# Autodesk Inventor assembly: 110033226_iam_14_內城堡
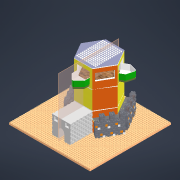
[picture p0: Inventor's stored thumbnail of the model, 180x180]
Saved by Autodesk Inventor 2022 (Build 260153000, 153)
## iProperties
Created: 2022-07-01
Part Number: 110033226_iam_14_內城堡
Document SubType Name: Assembly
Designer: User
Author: User
## Documents named in this file (4)
- D:\D-disk\pomelo\大一\下學期\機械設計製圖\1100332260_LEGOproj_沒有公主城堡\110033226_iam_14_內城堡.iam
- D:\D-disk\pomelo\大一\下學期\機械設計製圖\1100332260_LEGOproj_沒有公主城堡\110033226_ipt_54_內城堡底座.ipt
- D:\D-disk\pomelo\大一\下學期\機械設計製圖\1100332260_LEGOproj_沒有公主城堡\110033226_ipt_54_內城堡中柱.ipt
- D:\D-disk\pomelo\大一\下學期\機械設計製圖\1100332260_LEGOproj_沒有公主城堡\110033226_ipt_34_中心城堡圍牆.ipt
## Components (14 placed, 3 different names)
1. 110033226_ipt_54_內城堡底座:1 — 貼合:1, 貼合:2, 貼合:3, 貼合:4, 角度:1, 貼合:5, 貼合:9, 貼合:12, 貼合:15, 貼合:18
2. 110033226_ipt_54_內城堡中柱:1 — 貼合:4, 角度:1, 貼合:5, 貼合:10, 貼合:11, 貼合:13, 貼合:14, 貼合:16, 貼合:17, 貼合:19, 貼合:20
3. 110033226_ipt_34_中心城堡圍牆:2 — 貼合:9, 貼合:10, 貼合:11
4. 110033226_ipt_34_中心城堡圍牆:5
5. 110033226_ipt_34_中心城堡圍牆:6
6. 110033226_ipt_34_中心城堡圍牆:1 — 貼合:12, 貼合:13, 貼合:14
7. 110033226_ipt_34_中心城堡圍牆:7
8. 110033226_ipt_34_中心城堡圍牆:8
9. 110033226_ipt_34_中心城堡圍牆:9 — 貼合:15, 貼合:16, 貼合:17
10. 110033226_ipt_34_中心城堡圍牆:10
11. 110033226_ipt_34_中心城堡圍牆:11
12. 110033226_ipt_34_中心城堡圍牆:12 — 貼合:18, 貼合:19, 貼合:20
13. 110033226_ipt_34_中心城堡圍牆:13
14. 110033226_ipt_34_中心城堡圍牆:14
## Component patterns: (3 elements, first: 110033226_ipt_34_中心城堡圍牆:2), (3 elements, first: 110033226_ipt_34_中心城堡圍牆:1), (3 elements, first: 110033226_ipt_34_中心城堡圍牆:9), (3 elements, first: 110033226_ipt_34_中心城堡圍牆:12)
## Relationships (18: Mate 17, Angle 1)
- 貼合:1 [Mate]: 110033226_ipt_54_內城堡底座:1
- 貼合:2 [Mate]: 110033226_ipt_54_內城堡底座:1
- 貼合:3 [Mate]: 110033226_ipt_54_內城堡底座:1
- 貼合:4 [Mate]: 110033226_ipt_54_內城堡底座:1 ↔ 110033226_ipt_54_內城堡中柱:1
- 角度:1 [Angle] (0 deg): 110033226_ipt_54_內城堡底座:1 ↔ 110033226_ipt_54_內城堡中柱:1
- 貼合:5 [Mate]: 110033226_ipt_54_內城堡底座:1 ↔ 110033226_ipt_54_內城堡中柱:1
- 貼合:9 [Mate]: 110033226_ipt_54_內城堡底座:1 ↔ 110033226_ipt_34_中心城堡圍牆:2
- 貼合:10 [Mate]: 110033226_ipt_54_內城堡中柱:1 ↔ 110033226_ipt_34_中心城堡圍牆:2
- 貼合:11 [Mate]: 110033226_ipt_54_內城堡中柱:1 ↔ 110033226_ipt_34_中心城堡圍牆:2
- 貼合:12 [Mate]: 110033226_ipt_54_內城堡底座:1 ↔ 110033226_ipt_34_中心城堡圍牆:1
- 貼合:13 [Mate]: 110033226_ipt_54_內城堡中柱:1 ↔ 110033226_ipt_34_中心城堡圍牆:1
- 貼合:14 [Mate]: 110033226_ipt_54_內城堡中柱:1 ↔ 110033226_ipt_34_中心城堡圍牆:1
- 貼合:15 [Mate]: 110033226_ipt_54_內城堡底座:1 ↔ 110033226_ipt_34_中心城堡圍牆:9
- 貼合:16 [Mate]: 110033226_ipt_54_內城堡中柱:1 ↔ 110033226_ipt_34_中心城堡圍牆:9
- 貼合:17 [Mate]: 110033226_ipt_54_內城堡中柱:1 ↔ 110033226_ipt_34_中心城堡圍牆:9
- 貼合:18 [Mate]: 110033226_ipt_54_內城堡底座:1 ↔ 110033226_ipt_34_中心城堡圍牆:12
- 貼合:19 [Mate]: 110033226_ipt_54_內城堡中柱:1 ↔ 110033226_ipt_34_中心城堡圍牆:12
- 貼合:20 [Mate]: 110033226_ipt_54_內城堡中柱:1 ↔ 110033226_ipt_34_中心城堡圍牆:12
